# Autodesk Inventor assembly: MTLV2 Frame
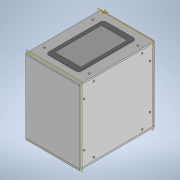
[picture p0: Inventor's stored thumbnail of the model, 180x180]
Saved by Autodesk Inventor 2020 (Build 240168000, 168)
## iProperties
Created: 2020-04-08
Part Number: MTLV2 Frame
Document SubType Name: Assembly
Designer: angusaitken
Author: angusaitken
## Documents named in this file (23)
- \\Mac\Home\Desktop\3D\MTLV2 Frame.iam
- \\Mac\Home\Downloads\5537T501_ALUMINUM T-SLOTTED FRAMING EXTRUSION.ipt
- \\Mac\Home\Downloads\5537T501_ALUMINUM T-SLOTTED FRAMING EXTRUSION_CPY.ipt
- \\Mac\Home\Downloads\5537T289_ALUMINUM T-SLOTTED FRAMING EXTRUSION.ipt
- \\Mac\Home\Downloads\5537T501_ALUMINUM T-SLOTTED FRAMING EXTRUSION_CPY_CPY.ipt
- \\Mac\Home\Downloads\5537T289_ALUMINUM T-SLOTTED FRAMING EXTRUSION_CPY.ipt
- \\Mac\Home\Downloads\5537T501_ALUMINUM T-SLOTTED FRAMING EXTRUSION_MIR.ipt
- \\Mac\Home\Downloads\5537T289_ALUMINUM T-SLOTTED FRAMING EXTRUSION_MIR.ipt
- \\Mac\Home\Downloads\5537T289_ALUMINUM T-SLOTTED FRAMING EXTRUSION_CPY_MIR.ipt
- \\Mac\Home\Downloads\5537T501_ALUMINUM T-SLOTTED FRAMING EXTRUSION_CPY1.ipt
- \\Mac\Home\Downloads\5537T501_ALUMINUM T-SLOTTED FRAMING EXTRUSION_CPY1_CPY.ipt
- \\Mac\Home\Downloads\5537T501_ALUMINUM T-SLOTTED FRAMING EXTRUSION_CPY1_CPY1.ipt
- \\Mac\Home\Downloads\5537T501_ALUMINUM T-SLOTTED FRAMING EXTRUSION_CPY1_CPY2.ipt
- \\Mac\Home\Downloads\5537T501_ALUMINUM T-SLOTTED FRAMING EXTRUSION_MIR1.ipt
- \\Mac\Home\Downloads\5537T501_ALUMINUM T-SLOTTED FRAMING EXTRUSION_CPY_MIR.ipt
- \\Mac\Home\Downloads\5537T289_ALUMINUM T-SLOTTED FRAMING EXTRUSION_MIR1.ipt
- \\Mac\Home\Downloads\5537T501_ALUMINUM T-SLOTTED FRAMING EXTRUSION_CPY_CPY_MIR.ipt
- \\Mac\Home\Downloads\5537T289_ALUMINUM T-SLOTTED FRAMING EXTRUSION_CPY_MIR1.ipt
- \\Mac\Home\Downloads\5537T501_ALUMINUM T-SLOTTED FRAMING EXTRUSION_MIR_MIR.ipt
- \\Mac\Home\Downloads\5537T289_ALUMINUM T-SLOTTED FRAMING EXTRUSION_CPY_MIR_MIR.ipt
- \\Mac\Home\Downloads\5537T289_ALUMINUM T-SLOTTED FRAMING EXTRUSION_MIR_MIR.ipt
- \\Mac\Home\Desktop\3D\Raspberry Pi 7 Touch Screen LCD.ipt
- \\Mac\Home\Desktop\3D\Front face.ipt
## Components (22 placed, 22 different names)
1. 5537T501_ALUMINUM T-SLOTTED FRAMING EXTRUSION:1 — Mate:1, Mate:3, Mate:4, Mate:20, Flush:5
2. 5537T501_ALUMINUM T-SLOTTED FRAMING EXTRUSION_CPY:1 — Flush:1, Mate:2, Flush:4
3. 5537T289_ALUMINUM T-SLOTTED FRAMING EXTRUSION:1 — Mate:1, Flush:1, Mate:2, Mate:12
4. 5537T501_ALUMINUM T-SLOTTED FRAMING EXTRUSION_CPY_CPY:1 — Mate:5, Mate:24, Mate:25
5. 5537T289_ALUMINUM T-SLOTTED FRAMING EXTRUSION_CPY:1 — Mate:3, Mate:4, Mate:5, Mate:9, Flush:2
6. 5537T501_ALUMINUM T-SLOTTED FRAMING EXTRUSION_MIR:1 — Mate:6, Mate:7, Mate:8
7. 5537T289_ALUMINUM T-SLOTTED FRAMING EXTRUSION_MIR:1 — Mate:6, Mate:11
8. 5537T289_ALUMINUM T-SLOTTED FRAMING EXTRUSION_CPY_MIR:1 — Mate:7, Mate:8, Mate:10, Mate:24, Mate:25
9. 5537T501_ALUMINUM T-SLOTTED FRAMING EXTRUSION_CPY1:1 — Mate:9, Flush:2, Mate:22
10. 5537T501_ALUMINUM T-SLOTTED FRAMING EXTRUSION_CPY1_CPY:1 — Mate:10
11. 5537T501_ALUMINUM T-SLOTTED FRAMING EXTRUSION_CPY1_CPY1:1 — Mate:12
12. 5537T501_ALUMINUM T-SLOTTED FRAMING EXTRUSION_CPY1_CPY2:1 — Mate:11
13. 5537T501_ALUMINUM T-SLOTTED FRAMING EXTRUSION_MIR1:1 — Mate:14, Mate:16, Mate:17
14. 5537T501_ALUMINUM T-SLOTTED FRAMING EXTRUSION_CPY_MIR:1 — Mate:13, Flush:3
15. 5537T289_ALUMINUM T-SLOTTED FRAMING EXTRUSION_MIR1:1 — Mate:13, Flush:3, Mate:14
16. 5537T501_ALUMINUM T-SLOTTED FRAMING EXTRUSION_CPY_CPY_MIR:1 — Mate:15
17. 5537T289_ALUMINUM T-SLOTTED FRAMING EXTRUSION_CPY_MIR1:1 — Mate:15, Mate:16, Mate:17, Mate:22
18. 5537T501_ALUMINUM T-SLOTTED FRAMING EXTRUSION_MIR_MIR:1 — Mate:18, Mate:19
19. 5537T289_ALUMINUM T-SLOTTED FRAMING EXTRUSION_CPY_MIR_MIR:1 — Mate:18, Mate:19
20. 5537T289_ALUMINUM T-SLOTTED FRAMING EXTRUSION_MIR_MIR:1
21. Raspberry Pi 7 Touch Screen LCD:1 — Flush:6, Flush:7, Mate:21
22. Front face:1 — Mate:20, Flush:4, Flush:5, Flush:6, Flush:7, Mate:21
## Relationships (31: Mate 24, Flush 7)
- Mate:1: 5537T501_ALUMINUM T-SLOTTED FRAMING EXTRUSION:1 ↔ 5537T289_ALUMINUM T-SLOTTED FRAMING EXTRUSION:1
- Flush:1: 5537T501_ALUMINUM T-SLOTTED FRAMING EXTRUSION_CPY:1 ↔ 5537T289_ALUMINUM T-SLOTTED FRAMING EXTRUSION:1
- Mate:2: 5537T501_ALUMINUM T-SLOTTED FRAMING EXTRUSION_CPY:1 ↔ 5537T289_ALUMINUM T-SLOTTED FRAMING EXTRUSION:1
- Mate:3: 5537T501_ALUMINUM T-SLOTTED FRAMING EXTRUSION:1 ↔ 5537T289_ALUMINUM T-SLOTTED FRAMING EXTRUSION_CPY:1
- Mate:4: 5537T501_ALUMINUM T-SLOTTED FRAMING EXTRUSION:1 ↔ 5537T289_ALUMINUM T-SLOTTED FRAMING EXTRUSION_CPY:1
- Mate:5: 5537T501_ALUMINUM T-SLOTTED FRAMING EXTRUSION_CPY_CPY:1 ↔ 5537T289_ALUMINUM T-SLOTTED FRAMING EXTRUSION_CPY:1
- Mate:6: 5537T501_ALUMINUM T-SLOTTED FRAMING EXTRUSION_MIR:1 ↔ 5537T289_ALUMINUM T-SLOTTED FRAMING EXTRUSION_MIR:1
- Mate:7: 5537T501_ALUMINUM T-SLOTTED FRAMING EXTRUSION_MIR:1 ↔ 5537T289_ALUMINUM T-SLOTTED FRAMING EXTRUSION_CPY_MIR:1
- Mate:8: 5537T501_ALUMINUM T-SLOTTED FRAMING EXTRUSION_MIR:1 ↔ 5537T289_ALUMINUM T-SLOTTED FRAMING EXTRUSION_CPY_MIR:1
- Mate:9: 5537T289_ALUMINUM T-SLOTTED FRAMING EXTRUSION_CPY:1 ↔ 5537T501_ALUMINUM T-SLOTTED FRAMING EXTRUSION_CPY1:1
- Flush:2: 5537T289_ALUMINUM T-SLOTTED FRAMING EXTRUSION_CPY:1 ↔ 5537T501_ALUMINUM T-SLOTTED FRAMING EXTRUSION_CPY1:1
- Mate:10: 5537T289_ALUMINUM T-SLOTTED FRAMING EXTRUSION_CPY_MIR:1 ↔ 5537T501_ALUMINUM T-SLOTTED FRAMING EXTRUSION_CPY1_CPY:1
- Mate:11: 5537T289_ALUMINUM T-SLOTTED FRAMING EXTRUSION_MIR:1 ↔ 5537T501_ALUMINUM T-SLOTTED FRAMING EXTRUSION_CPY1_CPY2:1
- Mate:12: 5537T289_ALUMINUM T-SLOTTED FRAMING EXTRUSION:1 ↔ 5537T501_ALUMINUM T-SLOTTED FRAMING EXTRUSION_CPY1_CPY1:1
- Mate:13: 5537T501_ALUMINUM T-SLOTTED FRAMING EXTRUSION_CPY_MIR:1 ↔ 5537T289_ALUMINUM T-SLOTTED FRAMING EXTRUSION_MIR1:1
- Flush:3: 5537T501_ALUMINUM T-SLOTTED FRAMING EXTRUSION_CPY_MIR:1 ↔ 5537T289_ALUMINUM T-SLOTTED FRAMING EXTRUSION_MIR1:1
- Mate:14: 5537T501_ALUMINUM T-SLOTTED FRAMING EXTRUSION_MIR1:1 ↔ 5537T289_ALUMINUM T-SLOTTED FRAMING EXTRUSION_MIR1:1
- Mate:15: 5537T501_ALUMINUM T-SLOTTED FRAMING EXTRUSION_CPY_CPY_MIR:1 ↔ 5537T289_ALUMINUM T-SLOTTED FRAMING EXTRUSION_CPY_MIR1:1
- Mate:16: 5537T501_ALUMINUM T-SLOTTED FRAMING EXTRUSION_MIR1:1 ↔ 5537T289_ALUMINUM T-SLOTTED FRAMING EXTRUSION_CPY_MIR1:1
- Mate:17: 5537T501_ALUMINUM T-SLOTTED FRAMING EXTRUSION_MIR1:1 ↔ 5537T289_ALUMINUM T-SLOTTED FRAMING EXTRUSION_CPY_MIR1:1
- Mate:18: 5537T501_ALUMINUM T-SLOTTED FRAMING EXTRUSION_MIR_MIR:1 ↔ 5537T289_ALUMINUM T-SLOTTED FRAMING EXTRUSION_CPY_MIR_MIR:1
- Mate:19: 5537T501_ALUMINUM T-SLOTTED FRAMING EXTRUSION_MIR_MIR:1 ↔ 5537T289_ALUMINUM T-SLOTTED FRAMING EXTRUSION_CPY_MIR_MIR:1
- Mate:20: 5537T501_ALUMINUM T-SLOTTED FRAMING EXTRUSION:1 ↔ Front face:1
- Flush:4 (-4.75 mm): 5537T501_ALUMINUM T-SLOTTED FRAMING EXTRUSION_CPY:1 ↔ Front face:1
- Flush:5 (-4.75 mm): 5537T501_ALUMINUM T-SLOTTED FRAMING EXTRUSION:1 ↔ Front face:1
- Flush:6 (34.62 mm): Raspberry Pi 7 Touch Screen LCD:1 ↔ Front face:1
- Flush:7 (1 mm): Raspberry Pi 7 Touch Screen LCD:1 ↔ Front face:1
- Mate:21 (25 mm): Raspberry Pi 7 Touch Screen LCD:1 ↔ Front face:1
- Mate:22: 5537T501_ALUMINUM T-SLOTTED FRAMING EXTRUSION_CPY1:1 ↔ 5537T289_ALUMINUM T-SLOTTED FRAMING EXTRUSION_CPY_MIR1:1
- Mate:24: 5537T501_ALUMINUM T-SLOTTED FRAMING EXTRUSION_CPY_CPY:1 ↔ 5537T289_ALUMINUM T-SLOTTED FRAMING EXTRUSION_CPY_MIR:1
- Mate:25: 5537T501_ALUMINUM T-SLOTTED FRAMING EXTRUSION_CPY_CPY:1 ↔ 5537T289_ALUMINUM T-SLOTTED FRAMING EXTRUSION_CPY_MIR:1
